# Autodesk Inventor assembly: Rebuild good piston - R
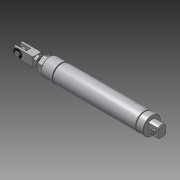
[picture p0: Inventor's stored thumbnail of the model, 180x180]
Saved by Autodesk Inventor 2014 SP1 (Build 180222100, 222)
## iProperties
Created: 2013-03-16
Part Number: Rebuild good piston - R
Document SubType Name: Assembly
Designer: Arpan
Mass: 1031.9 g
Surface Area: 880.309 cm^2
Volume: 144.619 cm^3
Density: 7.13533 g/cm^3
Author: Arpan
## Documents named in this file (12)
- C:\Users\Moses\Documents\Inventor\Sally Rebuild\Rebuild Sally\Rebuild good piston - R.iam
- C:\Users\Moses\Documents\Inventor\Sally Rebuild\Rebuild Sally\176_DP_D_229__F_D_231_1__F_D_3556__2_03\1.ipt
- C:\Users\Moses\Documents\Inventor\Sally Rebuild\Rebuild Sally\176_DP_D_229__F_D_231_1__F_D_3556__2_03\2.ipt
- C:\Users\Moses\Documents\Inventor\Sally Rebuild\Rebuild Sally\176_DP_D_229__F_D_231_1__F_D_3556__2_03\3.ipt
- C:\Users\Moses\Documents\Inventor\Sally Rebuild\Rebuild Sally\176_DP_D_229__F_D_231_1__F_D_3556__2_03\4.ipt
- C:\Users\Moses\Documents\Inventor\Sally Rebuild\Rebuild Sally\176_DP_D_229__F_D_231_1__F_D_3556__2_03\7.ipt
- C:\Users\Moses\Documents\Inventor\Sally Rebuild\Rebuild Sally\176_DP_D_229__F_D_231_1__F_D_3556__2_03\8.ipt
- C:\Users\Moses\Documents\Inventor\Sally Rebuild\Rebuild Sally\176_DP_D_229__F_D_231_1__F_D_3556__2_03\9.ipt
- C:\Users\Moses\Documents\Inventor\Sally Rebuild\Rebuild Sally\176_DP_D_229__F_D_231_1__F_D_3556__2_03\10.ipt
- C:\Users\Moses\Documents\Inventor\Sally Rebuild\Rebuild Sally\176_DP_D_229__F_D_231_1__F_D_3556__2_03\11.ipt
- C:\Users\Moses\Documents\Inventor\Sally Rebuild\Rebuild Sally\176_DP_D_229__F_D_231_1__F_D_3556__2_03\12.ipt
- C:\Users\Moses\Documents\Inventor\Sally Rebuild\Rebuild Sally\176_DP_D_229__F_D_231_1__F_D_3556__2_03\13.ipt
## Components (11 placed, 11 different names)
1. 1:1 — Mate:1, Mate:3, Mate:4, Flush:1, Mate:5, Angle:3, Angle:4
2. 2:1 — Mate:14
3. 3:1 — Mate:2, Mate:3, Mate:15, Flush:4
4. 4:1 — Mate:15, Angle:4, Flush:4
5. 7:1 — Flush:1, Mate:5, Angle:2, Angle:3
6. 8:1 — Mate:1, Mate:2, Mate:4, Mate:7, Mate:8, Flush:2, Mate:14
7. 9:1 — Mate:6, Angle:1, Mate:8, Flush:2, Mate:9, Flush:3, Mate:12, Mate:13
8. 10:1 — Mate:9, Flush:3, Mate:10, Mate:11
9. 11:1 — Mate:10, Mate:12
10. 12:1 — Mate:11, Mate:13
11. 13:1 — Mate:6, Mate:7, Angle:1, Angle:2
## Relationships (23: Mate 15, Flush 4, Angle 4)
- Mate:1: 1:1 ↔ 8:1
- Mate:2: 3:1 ↔ 8:1
- Mate:3 (174.752 mm): 1:1 ↔ 3:1
- Mate:4 (152.4 mm): 1:1 ↔ 8:1
- Flush:1 (2.8194 mm): 1:1 ↔ 7:1
- Mate:5: 1:1 ↔ 7:1
- Mate:6: 9:1 ↔ 13:1
- Mate:7: 8:1 ↔ 13:1
- Angle:1 (0 deg): 9:1 ↔ 13:1
- Angle:2 (0 deg): 7:1 ↔ 13:1
- Angle:3 (180 deg): 1:1 ↔ 7:1
- Mate:8: 8:1 ↔ 9:1
- Flush:2 (5.588 mm): 8:1 ↔ 9:1
- Mate:9: 9:1 ↔ 10:1
- Flush:3 (0.0635 mm): 9:1 ↔ 10:1
- Mate:10: 10:1 ↔ 11:1
- Mate:11: 10:1 ↔ 12:1
- Mate:12: 9:1 ↔ 11:1
- Mate:13: 9:1 ↔ 12:1
- Mate:14: 2:1 ↔ 8:1
- Mate:15: 3:1 ↔ 4:1
- Angle:4 (180 deg): 1:1 ↔ 4:1
- Flush:4 (-4.8641 mm): 3:1 ↔ 4:1
